# Autodesk Inventor assembly: #Spindexer
(part 2 of 2)
- Insert:222: PURCHASED,10-32x0.5in,BUTTONHEAD,BOLT:12 ↔ PLATE,SHOOTER,MOUNT:1
- Insert:223: PURCHASED,10-32x0.5in,BUTTONHEAD,BOLT:13 ↔ PLATE,SHOOTER,MOUNT:1
- Insert:224: PURCHASED,10-32x0.5in,BUTTONHEAD,BOLT:14 ↔ PLATE,SHOOTER,MOUNT:1
- Insert:225: PURCHASED,10-32x0.5in,BUTTONHEAD,BOLT:15 ↔ PLATE,SHOOTER,MOUNT:1
- Insert:226: PURCHASED,10-32x0.5in,BUTTONHEAD,BOLT:16 ↔ PLATE,SHOOTER,MOUNT:1
- Insert:227: PURCHASED,10-32x0.5in,BUTTONHEAD,BOLT:17 ↔ PLATE,SHOOTER,MOUNT:1
- Insert:228: PURCHASED,10-32x0.5in,BUTTONHEAD,BOLT:18 ↔ PLATE,SHOOTER,MOUNT:1
- Insert:229: PURCHASED,10-32x0.625in,BUTTONHEAD,BOLT:65 ↔ PLATE,KICKER,BACK:1
- Insert:230: PURCHASED,10-32x0.625in,BUTTONHEAD,BOLT:66 ↔ PLATE,KICKER,BACK:1
- Insert:232: PURCHASED,NYLOCK,10-32,NUT:6 ↔ CONTROLS,ENCODER,HEX_BORE:2
- Insert:233: PURCHASED,10-32x0.625in,BUTTONHEAD,BOLT:45 ↔ PLATE,SHOOTER,MOUNT:1
- Insert:234: PURCHASED,NYLOCK,10-32,NUT:5 ↔ CONTROLS,ENCODER,HEX_BORE:2
- Insert:235: PURCHASED,10-32x0.625in,BUTTONHEAD,BOLT:47 ↔ PLATE,SHOOTER,MOUNT:1
- Insert:236: PURCHASED,NYLOCK,10-32,NUT:8 ↔ CONTROLS,ENCODER,HEX_BORE:1
- Insert:238: PURCHASED,NYLOCK,10-32,NUT:7 ↔ CONTROLS,ENCODER,HEX_BORE:1
- Insert:239: PURCHASED,10-32x0.625in,FLATHEAD,BOLT:9 ↔ PLATE,SHOOTER,MOUNT:1
- Insert:240: PURCHASED,10-32x0.625in,FLATHEAD,BOLT:10 ↔ PLATE,SHOOTER,MOUNT:1
- Insert:241: PURCHASED,10-32x0.625in,FLATHEAD,BOLT:11 ↔ PLATE,SHOOTER,MOUNT:1
- Insert:242: PURCHASED,10-32x0.625in,FLATHEAD,BOLT:12 ↔ PLATE,SHOOTER,MOUNT:1
- Mate:152: PLATE,NUT-BLOCK,3-LONG:5 ↔ PLATE,SHOOTER,MOUNT:1
- Mate:153: PLATE,NUT-BLOCK,3-LONG:4 ↔ PLATE,SHOOTER,MOUNT:1
- Mate:154: STOCK,HEX,SHAFT,KICKER,BACK:1 ↔ STANDIN,BELT,70T,HTD5mm:1
- Mate:157: GEARBOX,VERSAPLANETARY,SINGLE-STAGE,HEX-SHAFT,0.5IN:1 ↔ PURCHASED,HEX_BEARING:10
- Mate:159: 3DPRINT,21T,HDT5mm,PULLEY:2 ↔ STOCK,HEX,SHAFT,KICKER,BACK:1
- Mate:160: 3DPRINT,24T,HTD5mm,PULLEY:1 ↔ STOCK,HEX,SHAFT,KICKER,BACK:1
- Mate:161: 3DPRINT,24T,HTD5mm,PULLEY:2 ↔ GEARBOX,VERSAPLANETARY,SINGLE-STAGE,HEX-SHAFT,0.5IN:1
- Mate:164: 3DPRINT,21T,HDT5mm,PULLEY:1 ↔ PLATE,KICKER,INSIDE:1
- Mate:165: STOCK,HEX,SHAFT,KICKER,BACK:1 ↔ PURCHASED,HEX_BEARING:11
- Flush:29: PURCHASED,HEX_BEARING:11 ↔ PURCHASED,HEX_BEARING:10
- Flush:30: 3DPRINT,KICKER,MOTOR,SPACER:1 ↔ GEARBOX,VERSAPLANETARY,SINGLE-STAGE,HEX-SHAFT,0.5IN:1
- Mate:166: 3DPRINT,KICKER,MOTOR,SPACER:1 ↔ GEARBOX,VERSAPLANETARY,SINGLE-STAGE,HEX-SHAFT,0.5IN:1
- Mate:168: STOCK,HEX,SHAFT,KICKER,FRONT:1 ↔ PURCHASED,GEAR,20DP,30T,HEX:2
- Mate:169: PLATE,KICKER,INSIDE:1 ↔ PURCHASED,GEAR,20DP,30T,HEX:1
- Insert:243: PLATE,KICKER,INSIDE:1 ↔ PURCHASED,HEX_BEARING:12
- Flush:31: PURCHASED,GEAR,20DP,30T,HEX:2 ↔ PURCHASED,GEAR,20DP,30T,HEX:1
- Mate:170: STOCK,HEX,SHAFT,KICKER,REVERSER:1 ↔ PURCHASED,GEAR,20DP,30T,HEX:1
- Mate:172: STOCK,HEX,SHAFT,KICKER,REVERSER:1 ↔ PURCHASED,HEX_BEARING:13
- Mate:173 (0.7937 mm): 3DPRINT,24T,HTD5mm,PULLEY:1 ↔ PURCHASED,HEX_BEARING:3
- Mate:177: 3DPRINT,21T,HDT5mm,PULLEY:2 ↔ PURCHASED,HEX_BEARING:11
- Mate:178: 3DPRINT,24T,HTD5mm,PULLEY:1 ↔ 3DPRINT,21T,HDT5mm,PULLEY:2
- Mate:179: PURCHASED,HEX_BEARING:12 ↔ PURCHASED,GEAR,20DP,30T,HEX:1
- Mate:180: 3DPRINT,21T,HDT5mm,PULLEY:1 ↔ PURCHASED,GEAR,20DP,30T,HEX:1
- Mate:181: 3DPRINT,21T,HDT5mm,PULLEY:1 ↔ PURCHASED,HEX_BEARING:13
- Mate:182: 3DPRINT,KICKER,MOTOR,SPACER:1 ↔ 3DPRINT,24T,HTD5mm,PULLEY:2
- Mate:183: 3DPRINT,KICKER,MOTOR,SUPPORT-PLATE,SPACER:1 ↔ GEARBOX,VERSAPLANETARY,SINGLE-STAGE,HEX-SHAFT,0.5IN:1
- Mate:184: 3DPRINT,KICKER,MOTOR,SUPPORT-PLATE,SPACER:1 ↔ 3DPRINT,24T,HTD5mm,PULLEY:2
- Mate:185: PLATE,KICKER,MOTOR,SUPPORT:1 ↔ STOCK,HEX,SHAFT,KICKER,BACK:1
- Mate:186: PLATE,KICKER,MOTOR,SUPPORT:1 ↔ GEARBOX,VERSAPLANETARY,SINGLE-STAGE,HEX-SHAFT,0.5IN:1
- Mate:187: PLATE,KICKER,MOTOR,SUPPORT:1 ↔ PURCHASED,HEX_BEARING:10
- Mate:188: PURCHASED,10-32x0.25in,BUTTONHEAD,BOLT:1 ↔ PLATE,KICKER,MOTOR,SUPPORT:1
- Mate:189: PURCHASED,10-32x0.25in,BUTTONHEAD,BOLT:2 ↔ PLATE,KICKER,MOTOR,SUPPORT:1
- Mate:190: PURCHASED,10-32x0.25in,BUTTONHEAD,BOLT:2 ↔ PURCHASED,HEX_BEARING:10
- Mate:191: PURCHASED,10-32x0.25in,BUTTONHEAD,BOLT:1 ↔ PURCHASED,HEX_BEARING:11
- Mate:192: STANDIN,BELT,70T,HTD5mm:1 ↔ GEARBOX,VERSAPLANETARY,SINGLE-STAGE,HEX-SHAFT,0.5IN:1
- Mate:193 (0.5 mm): 3DPRINT,24T,HTD5mm,PULLEY:2 ↔ STANDIN,BELT,70T,HTD5mm:1
- Mate:194: STOCK,HEX,SHAFT,KICKER,REVERSER:1 ↔ STANDIN,BELT,85T,HTD5mm:1
- Mate:195: STOCK,HEX,SHAFT,KICKER,BACK:1 ↔ STANDIN,BELT,85T,HTD5mm:1
- Mate:196 (0.5 mm): 3DPRINT,21T,HDT5mm,PULLEY:2 ↔ STANDIN,BELT,85T,HTD5mm:1
- Mate:197: PLATE,REVERSER,SUPPORT:1 ↔ PURCHASED,HEX_BEARING:13
- Mate:198: PLATE,KICKER,INSIDE:1 ↔ PLATE,REVERSER,SUPPORT:1
- Mate:199: PLATE,KICKER,INSIDE:1 ↔ PLATE,REVERSER,SUPPORT:1
- Insert:244: PLATE,KICKER,INSIDE:1 ↔ STOCK,REVERSER,STANDOFF:1
- Insert:245: PLATE,KICKER,INSIDE:1 ↔ STOCK,REVERSER,STANDOFF:2
- Insert:246: PLATE,KICKER,INSIDE:1 ↔ STOCK,REVERSER,STANDOFF:3
- Insert:247: PURCHASED,10-32x0.5in,BUTTONHEAD,BOLT:19 ↔ PLATE,REVERSER,SUPPORT:1
- Insert:248: PURCHASED,10-32x0.5in,BUTTONHEAD,BOLT:20 ↔ PLATE,REVERSER,SUPPORT:1
- Insert:249: PURCHASED,10-32x0.5in,BUTTONHEAD,BOLT:21 ↔ PLATE,REVERSER,SUPPORT:1
- Insert:250: PURCHASED,10-32x0.5in,BUTTONHEAD,BOLT:22 ↔ PLATE,KICKER,INSIDE:1
- Insert:251: PURCHASED,10-32x0.5in,BUTTONHEAD,BOLT:23 ↔ PLATE,KICKER,INSIDE:1
- Insert:252: PURCHASED,10-32x0.5in,BUTTONHEAD,BOLT:24 ↔ PLATE,KICKER,INSIDE:1
- [Insert]: PURCHASED,WASHER,10-32:14 ↔ PURCHASED,10-32x0.625in,BUTTONHEAD,BOLT:67
- [Insert]: PURCHASED,WASHER,10-32:15 ↔ PURCHASED,10-32x0.625in,BUTTONHEAD,BOLT:68
- [Insert]: PURCHASED,WASHER,10-32:16 ↔ PURCHASED,10-32x0.625in,BUTTONHEAD,BOLT:69
- [Insert]: PURCHASED,WASHER,10-32:17 ↔ PURCHASED,10-32x0.625in,BUTTONHEAD,BOLT:70
- Insert:257: PURCHASED,WASHER,10-32:14 ↔ STOCK,HEX,SHAFT,KICKER,FRONT:1
- Insert:258: PURCHASED,WASHER,10-32:15 ↔ STOCK,HEX,SHAFT,KICKER,REVERSER:1
- Insert:259: PURCHASED,WASHER,10-32:16 ↔ STOCK,HEX,SHAFT,KICKER,BACK:1
- Insert:260: PURCHASED,WASHER,10-32:17 ↔ PURCHASED,HEX_BEARING:10
- [Insert]: PURCHASED,WASHER,10-32:18 ↔ PURCHASED,10-32x0.625in,BUTTONHEAD,BOLT:71
- [Insert]: PURCHASED,WASHER,10-32:19 ↔ PURCHASED,10-32x0.625in,BUTTONHEAD,BOLT:72
- Insert:263: PURCHASED,WASHER,10-32:19 ↔ STOCK,HEX,SHAFT,KICKER,BACK:1
- Insert:264: PURCHASED,WASHER,10-32:18 ↔ STOCK,HEX,SHAFT,KICKER,FRONT:1
- Mate:202: 3DPRINT,CABLE-SHROUD,QUARTER:1 ↔ PLATE,SHOOTER,MOUNT:1
- Mate:203: 3DPRINT,CABLE-SHROUD,QUARTER:1 ↔ PLATE,SHOOTER,MOUNT:1
- Mate:204: 3DPRINT,CABLE-SHROUD,QUARTER:1 ↔ PLATE,SHOOTER,MOUNT:1
- Mate:205: 3DPRINT,CABLE-SHROUD,QUARTER:2 ↔ 3DPRINT,CABLE-SHROUD,QUARTER:1
- Mate:206: 3DPRINT,CABLE-SHROUD,QUARTER:2 ↔ PLATE,SHOOTER,MOUNT:1
- Mate:207: 3DPRINT,CABLE-SHROUD,QUARTER:2 ↔ 3DPRINT,CABLE-SHROUD,QUARTER:1
- Mate:213: 3DPRINT,CABLE,TRAY,BL:1 ↔ PLATE,SHOOTER,MOUNT:1
- Mate:214: 3DPRINT,CABLE,TRAY,BL:1 ↔ PLATE,SHOOTER,MOUNT:1
- Flush:33: 3DPRINT,CABLE,TRAY,BL:1 ↔ 3DPRINT,CABLE-SHROUD,QUARTER:1
- Mate:215: 3DPRINT,CABLE,TRAY,BR:1 ↔ 3DPRINT,CABLE,TRAY,BL:1
- Mate:216: 3DPRINT,CABLE,TRAY,BR:1 ↔ 3DPRINT,CABLE,TRAY,BL:1
- Mate:217: 3DPRINT,CABLE,TRAY,TL:1 ↔ 3DPRINT,CABLE,TRAY,BR:1
- Mate:218: 3DPRINT,CABLE,TRAY,TL:1 ↔ 3DPRINT,CABLE,TRAY,BR:1
- Mate:219: 3DPRINT,CABLE,TRAY,TR:1 ↔ 3DPRINT,CABLE,TRAY,TL:1
- Mate:220: 3DPRINT,CABLE,TRAY,TR:1 ↔ 3DPRINT,CABLE,TRAY,TL:1
- Mate:222: PLATE,SHOOTER,MOUNT:1 ↔ PLATE,SHOOTER,SHEILD,LOWER:1
- Flush:34: PLATE,SHOOTER,MOUNT:1 ↔ PLATE,SHOOTER,SHEILD,LOWER:1
- Mate:223: 3DPRINT,CABLE-SHROUD,QUARTER:2 ↔ PLATE,SHOOTER,SHEILD,LOWER:1
- [Insert]: PURCHASED,10-32x0.625in,BUTTONHEAD,BOLT:73 ↔ PURCHASED,WASHER,10-32:20
- Insert:266: PURCHASED,WASHER,10-32:20 ↔ STOCK,HEX,SHAFT,KICKER,REVERSER:1
- Mate:224: 3DPRINT,TURRET,PINION,SHROUD:1 ↔ STOCK,HEX,SHAFT,TURRET,ENCODER:1
- Mate:225: 3DPRINT,TURRET,PINION,SHROUD:1 ↔ PLATE,SHOOTER,MOUNT:1
- Mate:226: 3DPRINT,TURRET,PINION,SHROUD:1 ↔ 3DPRINT,CABLE-SHROUD,QUARTER:2
- Insert:267: 3DPRINT,TURRET,PINION,SHROUD:1 ↔ PURCHASED,10-32x0.75in,BUTTONHEAD,BOLT:2
- Mate:227: 3DPRINT,TURRET,PINION,SHROUD,21T:1 ↔ STOCK,HEX,SHAFT,TURRET,DRIVE:1
- Mate:228: 3DPRINT,TURRET,PINION,SHROUD,21T:1 ↔ 3DPRINT,CABLE-SHROUD,QUARTER:1
- Mate:229: 3DPRINT,TURRET,PINION,SHROUD,21T:1 ↔ PLATE,SHOOTER,MOUNT:1
- Insert:268: PURCHASED,10-32x0.75in,BUTTONHEAD,BOLT:1 ↔ 3DPRINT,TURRET,PINION,SHROUD,21T:1
- Mate:231: PLATE,SHOOTER,MOUNT:1 ↔ PLATE,TURRET,MOTOR,MOUNT:1
- Insert:269: PLATE,TURRET,MOTOR,MOUNT:1 ↔ STOCK,CHURRO,HEX,TURRET,MOTOR-MOUNT,SPACER:3
- Insert:270: PURCHASED,0.25-20x0.5in,BUTTONHEAD,BOLT:5 ↔ PLATE,SHOOTER,MOUNT:1
- Mate:232: PURCHASED,10-32x0.75in,BUTTONHEAD,BOLT:1 ↔ CONTROLS,ENCODER,HEX_BORE:2
- Mate:233: PLATE,SHOOTER,MOUNT:1 ↔ PLATE,TURRET,MOTOR,MOUNT:2
- Mate:234: PLATE,SHOOTER,MOUNT:1 ↔ PLATE,TURRET,MOTOR,MOUNT:2
- Mate:235: PLATE,SHOOTER,MOUNT:1 ↔ PLATE,TURRET,MOTOR,MOUNT:2
- Insert:271: PLATE,TURRET,MOTOR,MOUNT:2 ↔ STOCK,CHURRO,HEX,TURRET,MOTOR-MOUNT,SPACER:4
- Insert:272: STOCK,CHURRO,HEX,TURRET,MOTOR-MOUNT,SPACER:7 ↔ PLATE,TURRET,MOTOR,MOUNT:2
- Insert:273: STOCK,CHURRO,HEX,TURRET,MOTOR-MOUNT,SPACER:8 ↔ PLATE,TURRET,MOTOR,MOUNT:2
- Insert:274: PLATE,SHOOTER,MOUNT:1 ↔ STOCK,CHURRO,HEX,TURRET,MOTOR-MOUNT,SPACER:4
- Insert:275: PLATE,TURRET,MOTOR,MOUNT:2 ↔ PURCHASED,HEX_BEARING:9
- Insert:276: PURCHASED,0.25-20x0.5in,BUTTONHEAD,BOLT:12 ↔ PLATE,SHOOTER,MOUNT:1
- Insert:277: PURCHASED,0.25-20x0.5in,BUTTONHEAD,BOLT:15 ↔ PLATE,TURRET,MOTOR,MOUNT:2
- Insert:278: PURCHASED,0.25-20x0.5in,BUTTONHEAD,BOLT:14 ↔ PLATE,TURRET,MOTOR,MOUNT:2
- Mate:236: PURCHASED,10-32x0.75in,BUTTONHEAD,BOLT:2 ↔ CONTROLS,ENCODER,HEX_BORE:1
- Insert:279: PURCHASED,0.25-20x0.5in,BUTTONHEAD,BOLT:16 ↔ PLATE,TURRET,MOTOR,MOUNT:2
- Insert:280: PURCHASED,0.25-20x0.5in,BUTTONHEAD,BOLT:17 ↔ PLATE,SHOOTER,MOUNT:1
- Insert:281: PURCHASED,0.25-20x0.5in,BUTTONHEAD,BOLT:18 ↔ PLATE,SHOOTER,MOUNT:1
- Insert:282: STOCK,CHURRO,HEX,TURRET,MOTOR-MOUNT,SUPPORT:1 ↔ PLATE,TURRET,MOTOR,MOUNT:1
- Mate:237: 3DPRINT,TURRET,LOCK:1 ↔ PLATE,SHOOTER,MOUNT:1
- Mate:238: 3DPRINT,TURRET,LOCK:1 ↔ PLATE,SHOOTER,MOUNT:1
- Flush:35: 3DPRINT,TURRET,LOCK:1 ↔ PLATE,TURRET,PINNION,GEAR:1
- Insert:283: STOCK,CHURRO,HEX,TURRET,LOCK:1 ↔ PLATE,SHOOTER,MOUNT:1
- Insert:284: STOCK,CHURRO,HEX,TURRET,LOCK:2 ↔ PLATE,SHOOTER,MOUNT:1
- Insert:285: 3DPRINT,TURRET,LOCK:1 ↔ PURCHASED,0.25-20x0.875in,SOCKETHEAD,BOLT:1
- Insert:286: 3DPRINT,TURRET,LOCK:1 ↔ PURCHASED,0.25-20x0.875in,SOCKETHEAD,BOLT:2
- Insert:287: PURCHASED,0.25-20x0.5in,BUTTONHEAD,BOLT:19 ↔ PLATE,SHOOTER,MOUNT:1
- Insert:288: PURCHASED,0.25-20x0.5in,BUTTONHEAD,BOLT:20 ↔ PLATE,SHOOTER,MOUNT:1
## Named parameters: d507_d407 = 0 mm, d508_d407 = 0 mm, d509_d407 = 0 mm, d510_d407 = 0 mm, d515_d407 = 0 mm, d516_d407 = 0 mm, d557_d515_d407 = 0 mm
